# Autodesk Inventor assembly: FrontMotorShaft
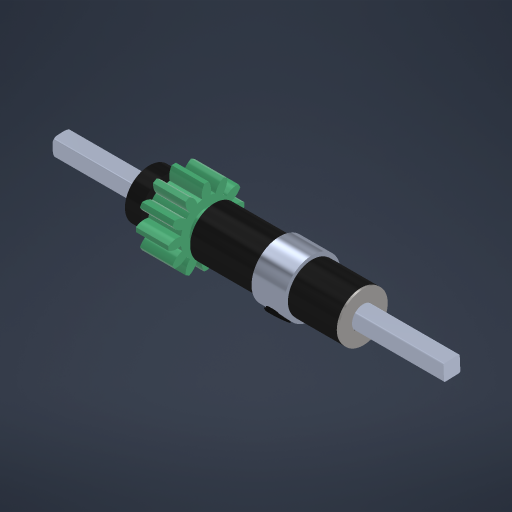
[picture p0: Inventor's stored thumbnail of the model, 512x512]
Saved by Autodesk Inventor 2023 (Build 270158000, 158)
## iProperties
Created: 2022-08-31
Part Number: FrontMotorShaft
Document SubType Name: Assembly
Designer: alex
Author: alex
## Documents named in this file (11)
- C:\Users\alex\Documents\GitHub\4067X_spin_up_cad\Chassis\IntermediateShaft.iam
- C:\Users\alex\Documents\GitHub\4067X_spin_up_cad\Library\Motion\Spacers\Spacer Nylon .375 OD\NSpacer .375 OD x .125.ipt
- C:\Users\alex\Documents\GitHub\4067X_spin_up_cad\Library\Motion\Spacers\Spacer Nylon .375 OD.ipt
- C:\Users\alex\Documents\GitHub\4067X_spin_up_cad\Library\Motion\Shaft Collar with Set Screw.ipt
- C:\Users\alex\Documents\GitHub\4067X_spin_up_cad\Library\Motion\Spacers\Spacer Nylon .375 OD\NSpacer .375 OD x .500.ipt
- C:\Users\alex\Documents\GitHub\4067X_spin_up_cad\Library\Motion\Shaft LS.ipt
- C:\Users\alex\Documents\GitHub\4067X_spin_up_cad\Library\Motion\Shaft LS\Shaft LS 3.0 in.ipt
- C:\Users\alex\Documents\GitHub\4067X_spin_up_cad\Library\Motion\Gears\12T Gear.ipt
- C:\Users\alex\Documents\GitHub\4067X_spin_up_cad\Library\Motion\Spacers\Spacer Nylon .375 OD\NSpacer .375 OD x .375.ipt
- C:\Users\alex\Documents\GitHub\4067X_spin_up_cad\Library\Motion\Spacers\Washer Steel\SWasher .375 OD x .015625.ipt
- C:\Users\alex\Documents\GitHub\4067X_spin_up_cad\Library\Motion\Spacers\Washer Steel.ipt
## Components (7 placed, 7 different names)
1. NSpacer .375 OD x .125:1 — Flush:1, Insert:6
2. Shaft LS 3.0 in:1 — Flush:1
3. 12T Gear:1 — Insert:6, Insert:10
4. NSpacer .375 OD x .375:3 — Insert:9, Insert:12
5. SWasher .375 OD x .015625:1 — Insert:9
6. Shaft Collar with Set Screw:1 — Insert:11, Insert:12
7. NSpacer .375 OD x .500:4 — Insert:10, Insert:11
## Relationships (6: Insert 5, Flush 1)
- Flush:1 (17.2641 mm): NSpacer .375 OD x .125:1 ↔ Shaft LS 3.0 in:1
- Insert:6: NSpacer .375 OD x .125:1 ↔ 12T Gear:1
- Insert:9: NSpacer .375 OD x .375:3 ↔ SWasher .375 OD x .015625:1
- Insert:10: 12T Gear:1 ↔ NSpacer .375 OD x .500:4
- Insert:11: Shaft Collar with Set Screw:1 ↔ NSpacer .375 OD x .500:4
- Insert:12: NSpacer .375 OD x .375:3 ↔ Shaft Collar with Set Screw:1
